# Autodesk Inventor assembly: PCB_Case
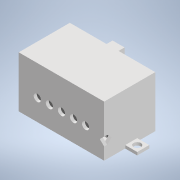
[picture p0: Inventor's stored thumbnail of the model, 180x180]
Saved by Autodesk Inventor 2021 (Build 250183000, 183)
## iProperties
Created: 2021-02-16
Part Number: PCB_Case
Document SubType Name: Assembly
Designer: Ryan
Author: Ryan
## Documents named in this file (4)
- C:\Users\Ryan\Documents\School\MQP\Case Model\PCB_Case.iam
- C:\Users\Ryan\Documents\School\MQP\Case Model\PCB_Case02.ipt
- C:\Users\Ryan\Documents\School\MQP\Case Model\PCB_Sheild.ipt
- C:\Users\Ryan\Documents\School\MQP\Case Model\PCB_Case02B.ipt
## Components (3 placed, 3 different names)
1. PCB_Case02:1 — Mate:1, Mate:2, Mate:3, Mate:4, Mate:5
2. PCB_Sheild:1 — Mate:1, Mate:2, Mate:3
3. PCB_Case02B:1 — Mate:4, Mate:5
## Relationships (5: Mate 5)
- Mate:1: PCB_Case02:1 ↔ PCB_Sheild:1
- Mate:2: PCB_Case02:1 ↔ PCB_Sheild:1
- Mate:3 (73.66 mm): PCB_Case02:1 ↔ PCB_Sheild:1
- Mate:4: PCB_Case02:1 ↔ PCB_Case02B:1
- Mate:5: PCB_Case02:1 ↔ PCB_Case02B:1
